# Autodesk Inventor assembly: 測定
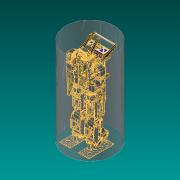
[picture p0: Inventor's stored thumbnail of the model, 180x180]
Saved by Autodesk Inventor 2016 (Build 200138000, 138)
## iProperties
Created: 2016-05-14
Part Number: 測定
Document SubType Name: Assembly
Designer: hiroaki
Author: hiroaki
## Documents named in this file (3)
- C:\Users\hiro\Documents\kenkyuu\二足\二足ver5.0\測定.iam
- C:\Users\hiro\Documents\kenkyuu\二足\二足ver5.0\本体.iam
- C:\Users\hiro\Documents\kenkyuu\二足\二足ver5.0\円柱.ipt
## Components (2 placed, 2 different names)
1. 本体:1 [sub-assembly] — フラッシュ:1, フラッシュ:2, フラッシュ:3, フラッシュ:4
2. 円柱:1 — フラッシュ:4
## Relationships (4: Flush 4)
- フラッシュ:1 [Flush]: 本体:1
- フラッシュ:2 [Flush]: 本体:1
- フラッシュ:3 [Flush]: 本体:1
- フラッシュ:4 [Flush]: 本体:1 ↔ 円柱:1
